# Autodesk Inventor assembly: batt support
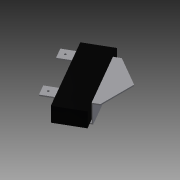
[picture p0: Inventor's stored thumbnail of the model, 180x180]
Saved by Autodesk Inventor 2015 (Build 190159000, 159)
## iProperties
Created: 2015-05-04
Part Number: batt support
Document SubType Name: Assembly
Designer: Kuba
Author: Kuba
## Documents named in this file (4)
- C:\Users\Kuba\Dysk Google\synergia\Synergolf\model\GOLF\batt support\batt support.iam
- C:\Users\Kuba\Dysk Google\synergia\Synergolf\model\GOLF\lipol_6000.ipt
- C:\Users\Kuba\Dysk Google\synergia\Synergolf\model\GOLF\batt support\dociskacz.ipt
- C:\Users\Kuba\Dysk Google\synergia\Synergolf\model\GOLF\batt support\batt-logic support.ipt
## Components (4 placed, 3 different names)
1. lipol_6000:1 — Równoległy:1, Zestawiający:1, Zestawiający:2, Zestawiający:3, Równoległy:2, Zestawiający:4
2. batt-logic support:1 — Zestawiający:3, Równoległy:2, Zestawiający:4
3. dociskacz:1 — Równoległy:1, Zestawiający:1, Zestawiający:2
4. dociskacz:2
## Component patterns: (2 elements, first: dociskacz:1)
## Relationships (6: Mate 4, Flush 2)
- Równoległy:1 [Flush]: lipol_6000:1 ↔ dociskacz:1
- Zestawiający:1 [Mate]: lipol_6000:1 ↔ dociskacz:1
- Zestawiający:2 [Mate] (-30 mm): lipol_6000:1 ↔ dociskacz:1
- Zestawiający:3 [Mate]: lipol_6000:1 ↔ batt-logic support:1
- Równoległy:2 [Flush]: lipol_6000:1 ↔ batt-logic support:1
- Zestawiający:4 [Mate]: lipol_6000:1 ↔ batt-logic support:1
